# Autodesk Inventor assembly: demo
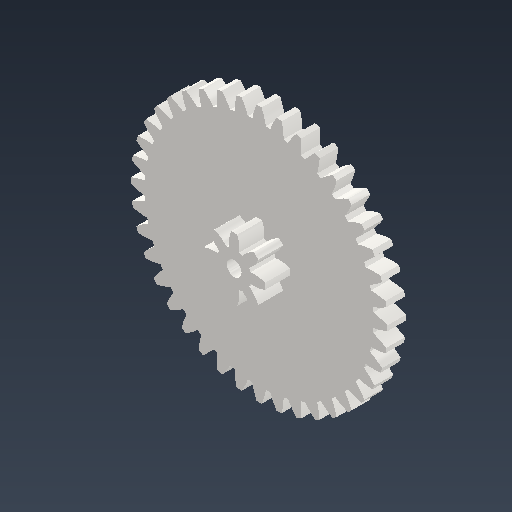
[picture p0: Inventor's stored thumbnail of the model, 512x512]
Saved by Autodesk Inventor 2025.3 (Build 293356000, 356)
## iProperties
Created: 2025-11-29
Part Number: demo
Document SubType Name: Assembly
Designer: 陳泓任
Author: 陳泓任
## Documents named in this file (3)
- C:\Users\Ou918\3D-model-temp\self-learning\gears\demo.iam
- C:\Users\Ou918\3D-model-temp\self-learning\gears\組合1\機械便覽魔法師\正齒輪21.ipt
- C:\Users\Ou918\3D-model-temp\self-learning\gears\組合1\機械便覽魔法師\正齒輪11.ipt
## Components (2 placed, 2 different names)
1. 正齒輪2:1 — 貼合:1, 貼合:2
2. 正齒輪1:1 — 貼合:1, 貼合:2
## Relationships (2: Mate 2)
- 貼合:1 [Mate]: 正齒輪2:1 ↔ 正齒輪1:1
- 貼合:2 [Mate]: 正齒輪2:1 ↔ 正齒輪1:1
